# Autodesk Inventor assembly: Default Motor Testbench
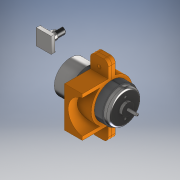
[picture p0: Inventor's stored thumbnail of the model, 180x180]
Saved by Autodesk Inventor 2018 (Build 220112000, 112)
## iProperties
Created: 2018-01-11
Part Number: Default Motor Testbench
Document SubType Name: Assembly
Designer: Moochster
Author: Moochster
## Documents named in this file (5)
- C:\Users\Moochster\OneDrive\Documents\2018 UBC\ELEC 391\Controller\CAD\Default Motor Testbench.iam
- C:\Users\Moochster\OneDrive\Documents\2018 UBC\ELEC 391\Controller\CAD\JD5B-2655W-R.ipt
- C:\Users\Moochster\OneDrive\Documents\2018 UBC\ELEC 391\Controller\CAD\PEC12R-4017F-N0024.iam
- C:\Users\Moochster\OneDrive\Documents\2018 UBC\ELEC 391\Controller\CAD\Motor Mount C-Clamp Top.ipt
- C:\Users\Moochster\OneDrive\Documents\2018 UBC\ELEC 391\Controller\CAD\Motor Mount C-Clamp Base.ipt
## Components (4 placed, 4 different names)
1. JD5B-2655W-R:1 — Mate:1, Mate:2, Angle:1
2. PEC12R-4017F-N0024:1 [sub-assembly]
3. Motor Mount C-Clamp Top:1 — Mate:1, Mate:4, Mate:5
4. Motor Mount C-Clamp Base:1 — Mate:2, Mate:3, Mate:4, Mate:5, Flush:1
## Relationships (7: Mate 5, Flush 1, Angle 1)
- Mate:1: JD5B-2655W-R:1 ↔ Motor Mount C-Clamp Top:1
- Mate:2: JD5B-2655W-R:1 ↔ Motor Mount C-Clamp Base:1
- Mate:3: Motor Mount C-Clamp Base:1
- Mate:4: Motor Mount C-Clamp Top:1 ↔ Motor Mount C-Clamp Base:1
- Mate:5: Motor Mount C-Clamp Top:1 ↔ Motor Mount C-Clamp Base:1
- Flush:1: Motor Mount C-Clamp Base:1
- Angle:1 (0 deg): JD5B-2655W-R:1
